# Autodesk Inventor assembly: Pino da correia
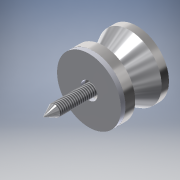
[picture p0: Inventor's stored thumbnail of the model, 180x180]
Saved by Autodesk Inventor 2016 (Build 200138000, 138)
## iProperties
Created: 2018-12-06
Part Number: Pino da correia
Document SubType Name: Assembly
Designer: dqm_r
Author: dqm_r
## Documents named in this file (4)
- C:\Users\dqm_r\OneDrive\Documentos\Inventor\Guitarra\Pino da correia.iam
- C:\Users\dqm_r\OneDrive\Documentos\Inventor\Guitarra\Peça 9.ipt
- C:\Users\dqm_r\OneDrive\Documentos\Inventor\Guitarra\Parafuso do Plug P10.ipt
- C:\Users\dqm_r\OneDrive\Documentos\Inventor\Guitarra\Arruela peça 9.ipt
## Components (3 placed, 3 different names)
1. Peça 9:1 — Insert:1, Rotational:1
2. Parafuso do Plug P10:1 — Insert:1
3. Arruela peça 9:1 — Rotational:1
## Relationships (2: Insert 1, RevoluteJoint 1)
- Insert:1: Peça 9:1 ↔ Parafuso do Plug P10:1
- Rotational:1 [RevoluteJoint]: Peça 9:1 ↔ Arruela peça 9:1
